# Autodesk Inventor assembly: Ensamble de estructura H
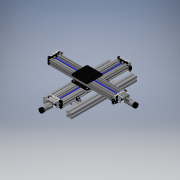
[picture p0: Inventor's stored thumbnail of the model, 180x180]
Saved by Autodesk Inventor 2018.3 (Build 223284000, 284)
## iProperties
Created: 2020-12-03
Part Number: Ensamble de estructura H
Material: Genérico
Description: STEP AP203
Document SubType Name: Assembly
Designer: SERGIO ROMO
Sending System: SolidWorks 2019
Preprocessor: SwSTEP 2.0
Title: Ensamble del Arreglo.STEP
Revision Number: ANY
## Documents named in this file (22)
- C:\Users\SERGIO ROMO\Documents\GitHub\RemBot\CAD\Balanceo de masa\Inventor\Ensamble de estructura H.iam
- C:\Users\SERGIO ROMO\Documents\GitHub\RemBot\CAD\Balanceo de masa\Inventor\C-Beam Actuator Lineal 500mm (Sin motor, sin carrito).ipt
- C:\Users\SERGIO ROMO\Documents\GitHub\RemBot\CAD\Balanceo de masa\Inventor\XLarge C-Beam Gantry Kit.iam
- C:\Users\SERGIO ROMO\Documents\GitHub\RemBot\CAD\Balanceo de masa\Inventor\Perfil de Aluminio.ipt
- C:\Users\SERGIO ROMO\Documents\GitHub\RemBot\CAD\Balanceo de masa\Inventor\Clavo.ipt
- C:\Users\SERGIO ROMO\Documents\GitHub\RemBot\CAD\Balanceo de masa\Inventor\Gearmotor_37D_19a1.ipt
- C:\Users\SERGIO ROMO\Documents\GitHub\RemBot\CAD\Balanceo de masa\Inventor\Impresion3D.ipt
- C:\Users\SERGIO ROMO\Documents\GitHub\RemBot\CAD\Balanceo de masa\Inventor\C-Beam Gantry Plate XLarge.step.ipt
- C:\Users\SERGIO ROMO\Documents\GitHub\RemBot\CAD\Balanceo de masa\Inventor\Bracket Inventor.ipt
- C:\Users\SERGIO ROMO\Documents\GitHub\RemBot\CAD\Balanceo de masa\Inventor\KW8-2.ipt
- C:\Users\SERGIO ROMO\Documents\GitHub\RemBot\CAD\Balanceo de masa\Inventor\Impresion3D sin Bracket.ipt
- C:\Users\SERGIO ROMO\Documents\GitHub\RemBot\CAD\Balanceo de masa\Inventor\Clavo de Arriba.ipt
- C:\Users\SERGIO ROMO\Documents\GitHub\RemBot\CAD\Balanceo de masa\Inventor\Tornillo final de carrera.ipt
- C:\Users\SERGIO ROMO\Documents\GitHub\RemBot\CAD\Balanceo de masa\Inventor\Perfil de Aluminio corta.ipt
- C:\Users\SERGIO ROMO\Documents\GitHub\RemBot\CAD\Balanceo de masa\Inventor\Triangulo.ipt
- C:\Users\SERGIO ROMO\Documents\GitHub\RemBot\CAD\Balanceo de masa\Inventor\TornilloM6.ipt
- C:\Users\SERGIO ROMO\Documents\GitHub\RemBot\CAD\Balanceo de masa\Inventor\Tuerca para tornilloM6.ipt
- C:\Users\SERGIO ROMO\Documents\GitHub\RemBot\CAD\Balanceo de masa\Inventor\Sujetador.ipt
- C:\Users\SERGIO ROMO\Documents\GitHub\RemBot\CAD\Balanceo de masa\Inventor\TornilloM8.ipt
- C:\Users\SERGIO ROMO\Documents\GitHub\RemBot\CAD\Balanceo de masa\Inventor\Tuerca para tornilloM8.ipt
- C:\Users\SERGIO ROMO\Documents\GitHub\RemBot\CAD\Balanceo de masa\Inventor\Tornillo para Bracket.ipt
- C:\Users\SERGIO ROMO\Documents\GitHub\RemBot\CAD\Balanceo de masa\Inventor\Tornillo para Motor Pololu.ipt
## Components (100 placed, 27 different names)
1. C-Beam Actuator Lineal 500mm (Sin motor, sin carrito)_1 — Coincidencia:6, Coincidencia:7, Coincidencia:8, Coincidencia:32, Coincidencia:33, Coincidencia:34, Coincidencia:35, Coincidencia:39, Coincidencia:41, Coincidencia:42, Coincidencia:45
2. XLarge C-Beam Gantry Kit_2 [sub-assembly] — Rígido:1
3. Perfil de Aluminio_4 — Coincidencia:32, Coincidencia:37, Coincidencia:44, Coincidencia:60, Coincidencia:61, Coincidencia:75, Coincidencia:77
4. Perfil de Aluminio_5 — Coincidencia:33, Coincidencia:36, Coincidencia:40, Coincidencia:64, Coincidencia:66, Coincidencia:79, Coincidencia:81
5. Clavo_8
6. Clavo_9
7. Gearmotor_37D_19a1_10 — Coincidencia:6
8. Gearmotor_37D_19a1_22
9. Impresion3D_28 — Coincidencia:1, Coincidencia:4, Coincidencia:15, Coincidencia:16, Coincidencia:28, Coincidencia:29, Coincidencia:30, Coincidencia:31, Coincidencia:83, Coincidencia:84
10. C-Beam Actuator Lineal 500mm (Sin motor, sin carrito):2 — Rígido:1, Coincidencia:2, Coincidencia:9, Coincidencia:10
11. C-Beam Gantry Plate XLarge.step:1
12. Bracket Inventor:1 — Coincidencia:1, Coincidencia:83, Coincidencia:84, Coincidencia:106, Coincidencia:107, Coincidencia:108, Coincidencia:109, Coincidencia:110, Coincidencia:111, Coincidencia:112, Coincidencia:113, Coincidencia:134, Coincidencia:135, Coincidencia:136, Coincidencia:137, Coincidencia:138, Coincidencia:139, Coincidencia:140, Coincidencia:141, Coincidencia:142, Coincidencia:143, Coincidencia:144, Coincidencia:145
13. Bracket Inventor:2 — Coincidencia:3, Coincidencia:11, Coincidencia:12, Coincidencia:85, Coincidencia:114, Coincidencia:115, Coincidencia:116, Coincidencia:117, Coincidencia:118, Coincidencia:119, Coincidencia:120, Coincidencia:121, Coincidencia:122, Coincidencia:123, Coincidencia:124, Coincidencia:125, Coincidencia:126, Coincidencia:127, Coincidencia:128, Coincidencia:129, Coincidencia:130, Coincidencia:131, Coincidencia:132, Coincidencia:133
14. Impresion3D:2 — Coincidencia:2, Coincidencia:3, Coincidencia:5, Coincidencia:11, Coincidencia:12, Coincidencia:13, Coincidencia:14, Coincidencia:24, Coincidencia:25, Coincidencia:26, Coincidencia:27, Coincidencia:85, Coincidencia:90, Coincidencia:91, Coincidencia:92, Coincidencia:93
15. KW8-2:1 — Coincidencia:4
16. KW8-2:2 — Coincidencia:5
17. KW8-2:3
18. KW8-2:4
19. Impresion3D sin Bracket:1 — Coincidencia:7, Coincidencia:8, Coincidencia:17, Coincidencia:18, Coincidencia:19, Coincidencia:86, Coincidencia:87, Coincidencia:88, Coincidencia:89
20. Impresion3D sin Bracket:2 — Coincidencia:9, Coincidencia:10, Coincidencia:20, Coincidencia:21, Coincidencia:22, Coincidencia:23, Coincidencia:94, Coincidencia:95, Coincidencia:96, Coincidencia:97
21. Clavo:3 — Coincidencia:13
22. Clavo:4 — Coincidencia:14
23. Clavo de Arriba:1 — Coincidencia:15
24. Clavo de Arriba:2 — Coincidencia:16
25. Clavo de Arriba:3 — Coincidencia:17
26. Clavo de Arriba:4 — Coincidencia:18, Coincidencia:19
27. Clavo de Arriba:5 — Coincidencia:21, Coincidencia:23
28. Clavo de Arriba:6 — Coincidencia:20, Coincidencia:22
29. Clavo de Arriba:7 — Coincidencia:24, Coincidencia:25
30. Clavo de Arriba:8 — Coincidencia:26, Coincidencia:27
31. Tornillo final de carrera:1 — Coincidencia:28, Coincidencia:30
32. Tornillo final de carrera:2 — Coincidencia:29, Coincidencia:31
33. Perfil de Aluminio corta:1 — Coincidencia:35, Coincidencia:37, Coincidencia:46, Coincidencia:55, Coincidencia:62, Coincidencia:63, Coincidencia:71, Coincidencia:72
34. Perfil de Aluminio corta:2 — Coincidencia:34, Coincidencia:36, Coincidencia:38, Coincidencia:43, Coincidencia:51, Coincidencia:56, Coincidencia:59, Coincidencia:65, Coincidencia:67, Coincidencia:68
35. Triangulo:1 — Coincidencia:40, Coincidencia:41, Coincidencia:47, Coincidencia:49, Coincidencia:102, Coincidencia:104
36. Triangulo:2 — Coincidencia:42, Coincidencia:43, Coincidencia:53, Coincidencia:98, Coincidencia:100
37. Triangulo:3 — Coincidencia:38, Coincidencia:39, Coincidencia:50, Coincidencia:103, Coincidencia:105
38. Triangulo:4 — Coincidencia:44, Coincidencia:45, Coincidencia:54, Coincidencia:99, Coincidencia:101
39. TornilloM6:1 — Coincidencia:46, Coincidencia:47, Coincidencia:48
40. Tuerca para tornilloM6:1 — Coincidencia:48, Coincidencia:49
41. TornilloM6:2 — Coincidencia:50, Coincidencia:51, Coincidencia:52
42. Tuerca para tornilloM6:2 — Coincidencia:52
43. TornilloM6:3 — Coincidencia:53, Coincidencia:56, Coincidencia:57
44. TornilloM6:4 — Coincidencia:54, Coincidencia:55, Coincidencia:58
45. Tuerca para tornilloM6:3 — Coincidencia:57
46. Tuerca para tornilloM6:4 — Coincidencia:58
47. Sujetador:1 — Coincidencia:59, Coincidencia:60
48. Sujetador:2 — Coincidencia:61, Coincidencia:62
49. Sujetador:3 — Coincidencia:65, Coincidencia:66
50. Sujetador:4 — Coincidencia:63, Coincidencia:64
51. TornilloM8:1 — Coincidencia:68, Coincidencia:70
52. TornilloM8:2 — Coincidencia:67, Coincidencia:69
53. Tuerca para tornilloM8:1 — Coincidencia:69
54. Tuerca para tornilloM8:2 — Coincidencia:70
55. TornilloM8:3 — Coincidencia:71, Coincidencia:74
56. TornilloM8:4 — Coincidencia:72, Coincidencia:73
57. Tuerca para tornilloM8:3 — Coincidencia:73
58. Tuerca para tornilloM8:4 — Coincidencia:74
59. TornilloM8:5 — Coincidencia:75, Coincidencia:76
60. TornilloM8:6 — Coincidencia:77, Coincidencia:78
61. Tuerca para tornilloM8:5 — Coincidencia:76
62. Tuerca para tornilloM8:6 — Coincidencia:78
63. TornilloM8:7 — Coincidencia:81, Coincidencia:82
64. TornilloM8:8 — Coincidencia:79, Coincidencia:80
65. Tuerca para tornilloM8:7 — Coincidencia:80
66. Tuerca para tornilloM8:8 — Coincidencia:82
67. Tornillo final de carrera:3 — Coincidencia:86, Coincidencia:88
68. Tornillo final de carrera:4 — Coincidencia:87, Coincidencia:89
69. Tornillo final de carrera:5 — Coincidencia:90, Coincidencia:92
70. Tornillo final de carrera:6 — Coincidencia:91, Coincidencia:93
71. Tornillo final de carrera:7 — Coincidencia:94, Coincidencia:96
72. Tornillo final de carrera:8 — Coincidencia:95, Coincidencia:97
73. TornilloM6:5 — Coincidencia:98
74. TornilloM6:6 — Coincidencia:99
75. Tuerca para tornilloM6:5 — Coincidencia:100
76. Tuerca para tornilloM6:6 — Coincidencia:101
77. TornilloM6:7 — Coincidencia:102
78. TornilloM6:8 — Coincidencia:103
79. Tuerca para tornilloM6:7 — Coincidencia:105
80. Tuerca para tornilloM6:8 — Coincidencia:104
81. Tornillo para Bracket:1 — Coincidencia:107, Coincidencia:111
82. Tornillo para Bracket:2 — Coincidencia:108, Coincidencia:112
83. Tornillo para Bracket:3 — Coincidencia:109, Coincidencia:110
84. Tornillo para Bracket:4 — Coincidencia:106, Coincidencia:113
85. Tornillo para Bracket:5 — Coincidencia:116, Coincidencia:121
86. Tornillo para Bracket:6 — Coincidencia:115, Coincidencia:118
87. Tornillo para Bracket:7 — Coincidencia:117, Coincidencia:120
88. Tornillo para Bracket:8 — Coincidencia:114, Coincidencia:119
89. Tornillo para Motor Pololu:1 — Coincidencia:127, Coincidencia:130
90. Tornillo para Motor Pololu:2 — Coincidencia:126, Coincidencia:128
91. Tornillo para Motor Pololu:3 — Coincidencia:124, Coincidencia:132
92. Tornillo para Motor Pololu:4 — Coincidencia:123, Coincidencia:131
93. Tornillo para Motor Pololu:5 — Coincidencia:125, Coincidencia:129
94. Tornillo para Motor Pololu:6 — Coincidencia:122, Coincidencia:133
95. Tornillo para Motor Pololu:7 — Coincidencia:138, Coincidencia:144
96. Tornillo para Motor Pololu:8 — Coincidencia:137, Coincidencia:143
97. Tornillo para Motor Pololu:9 — Coincidencia:136, Coincidencia:145
98. Tornillo para Motor Pololu:10 — Coincidencia:134, Coincidencia:141
99. Tornillo para Motor Pololu:11 — Coincidencia:135, Coincidencia:140
100. Tornillo para Motor Pololu:12 — Coincidencia:139, Coincidencia:142
## Relationships (146: Mate 145, WeldJoint 1)
- Rígido:1 [WeldJoint]: XLarge C-Beam Gantry Kit_2 ↔ C-Beam Actuator Lineal 500mm (Sin motor, sin carrito):2
- Coincidencia:1 [Mate]: Impresion3D_28 ↔ Bracket Inventor:1
- Coincidencia:2 [Mate]: C-Beam Actuator Lineal 500mm (Sin motor, sin carrito):2 ↔ Impresion3D:2
- Coincidencia:3 [Mate]: Bracket Inventor:2 ↔ Impresion3D:2
- Coincidencia:4 [Mate]: Impresion3D_28 ↔ KW8-2:1
- Coincidencia:5 [Mate]: Impresion3D:2 ↔ KW8-2:2
- Coincidencia:6 [Mate]: C-Beam Actuator Lineal 500mm (Sin motor, sin carrito)_1 ↔ Gearmotor_37D_19a1_10
- Coincidencia:7 [Mate]: C-Beam Actuator Lineal 500mm (Sin motor, sin carrito)_1 ↔ Impresion3D sin Bracket:1
- Coincidencia:8 [Mate]: C-Beam Actuator Lineal 500mm (Sin motor, sin carrito)_1 ↔ Impresion3D sin Bracket:1
- Coincidencia:9 [Mate]: C-Beam Actuator Lineal 500mm (Sin motor, sin carrito):2 ↔ Impresion3D sin Bracket:2
- Coincidencia:10 [Mate]: C-Beam Actuator Lineal 500mm (Sin motor, sin carrito):2 ↔ Impresion3D sin Bracket:2
- Coincidencia:11 [Mate]: Bracket Inventor:2 ↔ Impresion3D:2
- Coincidencia:12 [Mate]: Bracket Inventor:2 ↔ Impresion3D:2
- Coincidencia:13 [Mate]: Impresion3D:2 ↔ Clavo:3
- Coincidencia:14 [Mate]: Impresion3D:2 ↔ Clavo:4
- Coincidencia:15 [Mate]: Impresion3D_28 ↔ Clavo de Arriba:1
- Coincidencia:16 [Mate]: Impresion3D_28 ↔ Clavo de Arriba:2
- Coincidencia:17 [Mate]: Impresion3D sin Bracket:1 ↔ Clavo de Arriba:3
- Coincidencia:18 [Mate]: Impresion3D sin Bracket:1 ↔ Clavo de Arriba:4
- Coincidencia:19 [Mate]: Impresion3D sin Bracket:1 ↔ Clavo de Arriba:4
- Coincidencia:20 [Mate]: Impresion3D sin Bracket:2 ↔ Clavo de Arriba:6
- Coincidencia:21 [Mate]: Impresion3D sin Bracket:2 ↔ Clavo de Arriba:5
- Coincidencia:22 [Mate]: Impresion3D sin Bracket:2 ↔ Clavo de Arriba:6
- Coincidencia:23 [Mate]: Impresion3D sin Bracket:2 ↔ Clavo de Arriba:5
- Coincidencia:24 [Mate]: Impresion3D:2 ↔ Clavo de Arriba:7
- Coincidencia:25 [Mate]: Impresion3D:2 ↔ Clavo de Arriba:7
- Coincidencia:26 [Mate]: Impresion3D:2 ↔ Clavo de Arriba:8
- Coincidencia:27 [Mate]: Impresion3D:2 ↔ Clavo de Arriba:8
- Coincidencia:28 [Mate]: Impresion3D_28 ↔ Tornillo final de carrera:1
- Coincidencia:29 [Mate]: Impresion3D_28 ↔ Tornillo final de carrera:2
- Coincidencia:30 [Mate]: Impresion3D_28 ↔ Tornillo final de carrera:1
- Coincidencia:31 [Mate]: Impresion3D_28 ↔ Tornillo final de carrera:2
- Coincidencia:32 [Mate]: C-Beam Actuator Lineal 500mm (Sin motor, sin carrito)_1 ↔ Perfil de Aluminio_4
- Coincidencia:33 [Mate]: C-Beam Actuator Lineal 500mm (Sin motor, sin carrito)_1 ↔ Perfil de Aluminio_5
- Coincidencia:34 [Mate]: C-Beam Actuator Lineal 500mm (Sin motor, sin carrito)_1 ↔ Perfil de Aluminio corta:2
- Coincidencia:35 [Mate]: C-Beam Actuator Lineal 500mm (Sin motor, sin carrito)_1 ↔ Perfil de Aluminio corta:1
- Coincidencia:36 [Mate]: Perfil de Aluminio_5 ↔ Perfil de Aluminio corta:2
- Coincidencia:37 [Mate]: Perfil de Aluminio_4 ↔ Perfil de Aluminio corta:1
- Coincidencia:38 [Mate]: Perfil de Aluminio corta:2 ↔ Triangulo:3
- Coincidencia:39 [Mate]: C-Beam Actuator Lineal 500mm (Sin motor, sin carrito)_1 ↔ Triangulo:3
- Coincidencia:40 [Mate]: Perfil de Aluminio_5 ↔ Triangulo:1
- Coincidencia:41 [Mate]: C-Beam Actuator Lineal 500mm (Sin motor, sin carrito)_1 ↔ Triangulo:1
- Coincidencia:42 [Mate]: C-Beam Actuator Lineal 500mm (Sin motor, sin carrito)_1 ↔ Triangulo:2
- Coincidencia:43 [Mate]: Perfil de Aluminio corta:2 ↔ Triangulo:2
- Coincidencia:44 [Mate]: Perfil de Aluminio_4 ↔ Triangulo:4
- Coincidencia:45 [Mate]: C-Beam Actuator Lineal 500mm (Sin motor, sin carrito)_1 ↔ Triangulo:4
- Coincidencia:46 [Mate]: Perfil de Aluminio corta:1 ↔ TornilloM6:1
- Coincidencia:47 [Mate]: Triangulo:1 ↔ TornilloM6:1
- Coincidencia:48 [Mate]: TornilloM6:1 ↔ Tuerca para tornilloM6:1
- Coincidencia:49 [Mate]: Triangulo:1 ↔ Tuerca para tornilloM6:1
- Coincidencia:50 [Mate]: Triangulo:3 ↔ TornilloM6:2
- Coincidencia:51 [Mate]: Perfil de Aluminio corta:2 ↔ TornilloM6:2
- Coincidencia:52 [Mate]: TornilloM6:2 ↔ Tuerca para tornilloM6:2
- Coincidencia:53 [Mate]: Triangulo:2 ↔ TornilloM6:3
- Coincidencia:54 [Mate]: Triangulo:4 ↔ TornilloM6:4
- Coincidencia:55 [Mate]: Perfil de Aluminio corta:1 ↔ TornilloM6:4
- Coincidencia:56 [Mate]: Perfil de Aluminio corta:2 ↔ TornilloM6:3
- Coincidencia:57 [Mate]: TornilloM6:3 ↔ Tuerca para tornilloM6:3
- Coincidencia:58 [Mate]: TornilloM6:4 ↔ Tuerca para tornilloM6:4
- Coincidencia:59 [Mate]: Perfil de Aluminio corta:2 ↔ Sujetador:1
- Coincidencia:60 [Mate]: Perfil de Aluminio_4 ↔ Sujetador:1
- Coincidencia:61 [Mate]: Perfil de Aluminio_4 ↔ Sujetador:2
- Coincidencia:62 [Mate]: Perfil de Aluminio corta:1 ↔ Sujetador:2
- Coincidencia:63 [Mate]: Perfil de Aluminio corta:1 ↔ Sujetador:4
- Coincidencia:64 [Mate]: Perfil de Aluminio_5 ↔ Sujetador:4
- Coincidencia:65 [Mate]: Perfil de Aluminio corta:2 ↔ Sujetador:3
- Coincidencia:66 [Mate]: Perfil de Aluminio_5 ↔ Sujetador:3
- Coincidencia:67 [Mate]: Perfil de Aluminio corta:2 ↔ TornilloM8:2
- Coincidencia:68 [Mate]: Perfil de Aluminio corta:2 ↔ TornilloM8:1
- Coincidencia:69 [Mate]: TornilloM8:2 ↔ Tuerca para tornilloM8:1
- Coincidencia:70 [Mate]: TornilloM8:1 ↔ Tuerca para tornilloM8:2
- Coincidencia:71 [Mate]: Perfil de Aluminio corta:1 ↔ TornilloM8:3
- Coincidencia:72 [Mate]: Perfil de Aluminio corta:1 ↔ TornilloM8:4
- Coincidencia:73 [Mate]: TornilloM8:4 ↔ Tuerca para tornilloM8:3
- Coincidencia:74 [Mate]: TornilloM8:3 ↔ Tuerca para tornilloM8:4
- Coincidencia:75 [Mate]: Perfil de Aluminio_4 ↔ TornilloM8:5
- Coincidencia:76 [Mate]: TornilloM8:5 ↔ Tuerca para tornilloM8:5
- Coincidencia:77 [Mate]: Perfil de Aluminio_4 ↔ TornilloM8:6
- Coincidencia:78 [Mate]: TornilloM8:6 ↔ Tuerca para tornilloM8:6
- Coincidencia:79 [Mate]: Perfil de Aluminio_5 ↔ TornilloM8:8
- Coincidencia:80 [Mate]: TornilloM8:8 ↔ Tuerca para tornilloM8:7
- Coincidencia:81 [Mate]: Perfil de Aluminio_5 ↔ TornilloM8:7
- Coincidencia:82 [Mate]: TornilloM8:7 ↔ Tuerca para tornilloM8:8
- Coincidencia:83 [Mate]: Impresion3D_28 ↔ Bracket Inventor:1
- Coincidencia:84 [Mate]: Impresion3D_28 ↔ Bracket Inventor:1
- Coincidencia:85 [Mate]: Bracket Inventor:2 ↔ Impresion3D:2
- Coincidencia:86 [Mate]: Impresion3D sin Bracket:1 ↔ Tornillo final de carrera:3
- Coincidencia:87 [Mate]: Impresion3D sin Bracket:1 ↔ Tornillo final de carrera:4
- Coincidencia:88 [Mate]: Impresion3D sin Bracket:1 ↔ Tornillo final de carrera:3
- Coincidencia:89 [Mate]: Impresion3D sin Bracket:1 ↔ Tornillo final de carrera:4
- Coincidencia:90 [Mate]: Impresion3D:2 ↔ Tornillo final de carrera:5
- Coincidencia:91 [Mate]: Impresion3D:2 ↔ Tornillo final de carrera:6
- Coincidencia:92 [Mate]: Impresion3D:2 ↔ Tornillo final de carrera:5
- Coincidencia:93 [Mate]: Impresion3D:2 ↔ Tornillo final de carrera:6
- Coincidencia:94 [Mate]: Impresion3D sin Bracket:2 ↔ Tornillo final de carrera:7
- Coincidencia:95 [Mate]: Impresion3D sin Bracket:2 ↔ Tornillo final de carrera:8
- Coincidencia:96 [Mate]: Impresion3D sin Bracket:2 ↔ Tornillo final de carrera:7
- Coincidencia:97 [Mate]: Impresion3D sin Bracket:2 ↔ Tornillo final de carrera:8
- Coincidencia:98 [Mate]: Triangulo:2 ↔ TornilloM6:5
- Coincidencia:99 [Mate]: Triangulo:4 ↔ TornilloM6:6
- Coincidencia:100 [Mate]: Triangulo:2 ↔ Tuerca para tornilloM6:5
- Coincidencia:101 [Mate]: Triangulo:4 ↔ Tuerca para tornilloM6:6
- Coincidencia:102 [Mate]: Triangulo:1 ↔ TornilloM6:7
- Coincidencia:103 [Mate]: Triangulo:3 ↔ TornilloM6:8
- Coincidencia:104 [Mate]: Triangulo:1 ↔ Tuerca para tornilloM6:8
- Coincidencia:105 [Mate]: Triangulo:3 ↔ Tuerca para tornilloM6:7
- Coincidencia:106 [Mate]: Bracket Inventor:1 ↔ Tornillo para Bracket:4
- Coincidencia:107 [Mate]: Bracket Inventor:1 ↔ Tornillo para Bracket:1
- Coincidencia:108 [Mate]: Bracket Inventor:1 ↔ Tornillo para Bracket:2
- Coincidencia:109 [Mate]: Bracket Inventor:1 ↔ Tornillo para Bracket:3
- Coincidencia:110 [Mate]: Bracket Inventor:1 ↔ Tornillo para Bracket:3
- Coincidencia:111 [Mate]: Bracket Inventor:1 ↔ Tornillo para Bracket:1
- Coincidencia:112 [Mate]: Bracket Inventor:1 ↔ Tornillo para Bracket:2
- Coincidencia:113 [Mate]: Bracket Inventor:1 ↔ Tornillo para Bracket:4
- Coincidencia:114 [Mate]: Bracket Inventor:2 ↔ Tornillo para Bracket:8
- Coincidencia:115 [Mate]: Bracket Inventor:2 ↔ Tornillo para Bracket:6
- Coincidencia:116 [Mate]: Bracket Inventor:2 ↔ Tornillo para Bracket:5
- Coincidencia:117 [Mate]: Bracket Inventor:2 ↔ Tornillo para Bracket:7
- Coincidencia:118 [Mate]: Bracket Inventor:2 ↔ Tornillo para Bracket:6
- Coincidencia:119 [Mate]: Bracket Inventor:2 ↔ Tornillo para Bracket:8
- Coincidencia:120 [Mate]: Bracket Inventor:2 ↔ Tornillo para Bracket:7
- Coincidencia:121 [Mate]: Bracket Inventor:2 ↔ Tornillo para Bracket:5
- Coincidencia:122 [Mate]: Bracket Inventor:2 ↔ Tornillo para Motor Pololu:6
- Coincidencia:123 [Mate]: Bracket Inventor:2 ↔ Tornillo para Motor Pololu:4
- Coincidencia:124 [Mate]: Bracket Inventor:2 ↔ Tornillo para Motor Pololu:3
- Coincidencia:125 [Mate]: Bracket Inventor:2 ↔ Tornillo para Motor Pololu:5
- Coincidencia:126 [Mate]: Bracket Inventor:2 ↔ Tornillo para Motor Pololu:2
- Coincidencia:127 [Mate]: Bracket Inventor:2 ↔ Tornillo para Motor Pololu:1
- Coincidencia:128 [Mate]: Bracket Inventor:2 ↔ Tornillo para Motor Pololu:2
- Coincidencia:129 [Mate]: Bracket Inventor:2 ↔ Tornillo para Motor Pololu:5
- Coincidencia:130 [Mate]: Bracket Inventor:2 ↔ Tornillo para Motor Pololu:1
- Coincidencia:131 [Mate]: Bracket Inventor:2 ↔ Tornillo para Motor Pololu:4
- Coincidencia:132 [Mate]: Bracket Inventor:2 ↔ Tornillo para Motor Pololu:3
- Coincidencia:133 [Mate]: Bracket Inventor:2 ↔ Tornillo para Motor Pololu:6
- Coincidencia:134 [Mate]: Bracket Inventor:1 ↔ Tornillo para Motor Pololu:10
- Coincidencia:135 [Mate]: Bracket Inventor:1 ↔ Tornillo para Motor Pololu:11
- Coincidencia:136 [Mate]: Bracket Inventor:1 ↔ Tornillo para Motor Pololu:9
- Coincidencia:137 [Mate]: Bracket Inventor:1 ↔ Tornillo para Motor Pololu:8
- Coincidencia:138 [Mate]: Bracket Inventor:1 ↔ Tornillo para Motor Pololu:7
- Coincidencia:139 [Mate]: Bracket Inventor:1 ↔ Tornillo para Motor Pololu:12
- Coincidencia:140 [Mate]: Bracket Inventor:1 ↔ Tornillo para Motor Pololu:11
- Coincidencia:141 [Mate]: Bracket Inventor:1 ↔ Tornillo para Motor Pololu:10
- Coincidencia:142 [Mate]: Bracket Inventor:1 ↔ Tornillo para Motor Pololu:12
- Coincidencia:143 [Mate]: Bracket Inventor:1 ↔ Tornillo para Motor Pololu:8
- Coincidencia:144 [Mate]: Bracket Inventor:1 ↔ Tornillo para Motor Pololu:7
- Coincidencia:145 [Mate]: Bracket Inventor:1 ↔ Tornillo para Motor Pololu:9
